# Autodesk Inventor assembly: CuboidSecurityBoxCovered
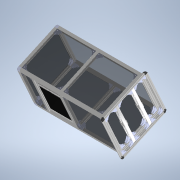
[picture p0: Inventor's stored thumbnail of the model, 180x180]
Saved by Autodesk Inventor 2021.1 (Build 251245010, 245A)
## iProperties
Created: 2020-11-09
Part Number: CuboidSecurityBoxCovered
Document SubType Name: Assembly
Designer: gisen
Author: gisen
## Documents named in this file (5)
- C:\Users\gisen\GitProjects\CAD-Data\CuboidAccessories\SecurityBox\CuboidSecurityBoxCovered.iam
- C:\Users\gisen\GitProjects\CAD-Data\CuboidAccessories\SecurityBox\Assemblies\CuboidSecurityBoxBasis.iam
- C:\Users\gisen\GitProjects\CAD-Data\GeneralComponentsTemplate\Fittings\BasicFrameBracket.ipt
- C:\Users\gisen\GitProjects\CAD-Data\CuboidAccessories\SecurityBox\Frames\BasicFrameCornerSide290.ipt
- C:\Users\gisen\GitProjects\CAD-Data\CuboidAccessories\SecurityBox\Plates\OutsideTopPlate_290_290.ipt
## Components (7 placed, 4 different names)
1. CuboidSecurityBoxBasis:1 [sub-assembly] — フラッシュ:1, フラッシュ:2, メイト:1, メイト:2, メイト:3, メイト:4, メイト:5, メイト:6, メイト:7, メイト:9, メイト:12, メイト:13, フラッシュ:3, メイト:14
2. BasicFrameBracket:1 — メイト:11, メイト:12, メイト:13
3. BasicFrameCornerSide290:1 — フラッシュ:1, フラッシュ:2, メイト:1, メイト:8, メイト:10, メイト:11, メイト:15
4. BasicFrameBracket:2 — メイト:8, メイト:9, メイト:10
5. BasicFrameBracket:3 — メイト:5, メイト:6, メイト:7
6. BasicFrameBracket:4 — メイト:2, メイト:3, メイト:4
7. OutsideTopPlate_290_290:1 — フラッシュ:3, メイト:14, メイト:15
## Relationships (18: Mate 15, Flush 3)
- フラッシュ:1 [Flush]: CuboidSecurityBoxBasis:1 ↔ BasicFrameCornerSide290:1
- フラッシュ:2 [Flush]: CuboidSecurityBoxBasis:1 ↔ BasicFrameCornerSide290:1
- メイト:1 [Mate]: CuboidSecurityBoxBasis:1 ↔ BasicFrameCornerSide290:1
- メイト:2 [Mate]: CuboidSecurityBoxBasis:1 ↔ BasicFrameBracket:4
- メイト:3 [Mate] (-10 mm): CuboidSecurityBoxBasis:1 ↔ BasicFrameBracket:4
- メイト:4 [Mate]: CuboidSecurityBoxBasis:1 ↔ BasicFrameBracket:4
- メイト:5 [Mate]: CuboidSecurityBoxBasis:1 ↔ BasicFrameBracket:3
- メイト:6 [Mate] (-10 mm): CuboidSecurityBoxBasis:1 ↔ BasicFrameBracket:3
- メイト:7 [Mate]: CuboidSecurityBoxBasis:1 ↔ BasicFrameBracket:3
- メイト:8 [Mate]: BasicFrameCornerSide290:1 ↔ BasicFrameBracket:2
- メイト:9 [Mate]: CuboidSecurityBoxBasis:1 ↔ BasicFrameBracket:2
- メイト:10 [Mate] (-10 mm): BasicFrameCornerSide290:1 ↔ BasicFrameBracket:2
- メイト:11 [Mate]: BasicFrameBracket:1 ↔ BasicFrameCornerSide290:1
- メイト:12 [Mate]: CuboidSecurityBoxBasis:1 ↔ BasicFrameBracket:1
- メイト:13 [Mate] (-10 mm): CuboidSecurityBoxBasis:1 ↔ BasicFrameBracket:1
- フラッシュ:3 [Flush]: CuboidSecurityBoxBasis:1 ↔ OutsideTopPlate_290_290:1
- メイト:14 [Mate]: CuboidSecurityBoxBasis:1 ↔ OutsideTopPlate_290_290:1
- メイト:15 [Mate]: BasicFrameCornerSide290:1 ↔ OutsideTopPlate_290_290:1
